# Autodesk Inventor assembly: wheel
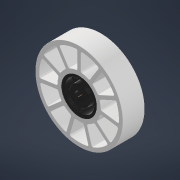
[picture p0: Inventor's stored thumbnail of the model, 180x180]
Saved by Autodesk Inventor 2022 (Build 260153000, 153)
## iProperties
Created: 2019-10-29
Part Number: wheel
Material: Green Stuff
Description: STEP AP203
Document SubType Name: Assembly
Designer: zehrab
Sending System: SolidWorks 2019
Preprocessor: SwSTEP 2.0
Title: am-3562 4IN 375Hex Bore Compliant Wheel.STEP
Revision Number: ANY
## Documents named in this file (3)
- C:\Users\zehrab\Documents\Inventor\Duck Carousel\wheel.iam
- C:\Users\zehrab\Documents\Inventor\Duck Carousel\4IN Compliant Wheel FINAL Overmold.ipt
- C:\Users\zehrab\Documents\Inventor\Duck Carousel\2in Wheel Intergrated 0375 HEX Hub.ipt
## Components (2 placed, 2 different names)
1. 4IN Compliant Wheel FINAL Overmold_1 — Mate:1
2. 2in Wheel Intergrated 0375 HEX Hub_2
## Relationships (1: Mate 1)
- Mate:1: 4IN Compliant Wheel FINAL Overmold_1
